# Autodesk Inventor assembly: magnet assembly
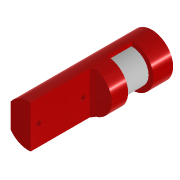
[picture p0: Inventor's stored thumbnail of the model, 180x180]
Saved by Autodesk Inventor 2022 (Build 260153000, 153)
## iProperties
Created: 2022-02-16
Part Number: magnet assembly
Document SubType Name: Assembly
Designer: piers
Author: piers
## Documents named in this file (3)
- C:\Users\piers\OneDrive\Documents\Inventor\Robotics Project\magnet assembly.iam
- C:\Users\piers\OneDrive\Documents\Inventor\Robotics Project\Tapered guide.ipt
- C:\Users\piers\OneDrive\Documents\Inventor\Robotics Project\Magnet.ipt
## Components (2 placed, 2 different names)
1. Tapered guide:1 — Mate:1, Mate:2, Mate:3, Mate:4, Mate:5
2. Magnet:1 — Mate:4, Mate:5
## Relationships (5: Mate 5)
- Mate:1: Tapered guide:1
- Mate:2: Tapered guide:1
- Mate:3: Tapered guide:1
- Mate:4: Tapered guide:1 ↔ Magnet:1
- Mate:5: Tapered guide:1 ↔ Magnet:1
